# Autodesk Inventor assembly: electronic_board
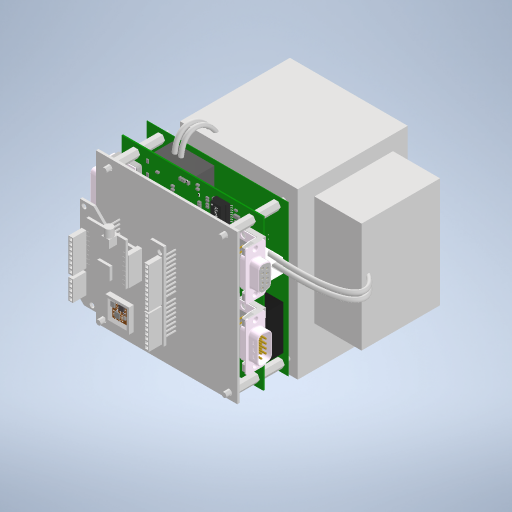
[picture p0: Inventor's stored thumbnail of the model, 512x512]
Saved by Autodesk Inventor 2023 (Build 270158000, 158)
## iProperties
Created: 2023-03-23
Part Number: electronic_board
Document SubType Name: Assembly
Designer: 310611102
Author: 310611102
## Documents named in this file (9)
- C:\Users\310611102\Documents\Inventor\SSR\avionics_2023ver\electronics\electronic_board.iam
- C:\Users\310611102\Documents\Inventor\SSR\avionics_2023ver\electronics\STM32 Communication Board ver1.0.ipt
- C:\Users\310611102\Documents\Inventor\SSR\avionics_2023ver\electronics\Power supply board.ipt
- C:\Users\310611102\Documents\Inventor\SSR\avionics_2023ver\electronics\copper_pillar_M3_L15.ipt
- C:\Users\310611102\Documents\Inventor\SSR\avionics_2023ver\electronics\battery_24V.ipt
- C:\Users\310611102\Documents\Inventor\SSR\avionics_2023ver\electronics\battery_5V.ipt
- C:\Users\310611102\Documents\Inventor\SSR\avionics_2023ver\electronics\MTI-7\MTi 1-series v3.iam
- C:\Users\310611102\Documents\Inventor\SSR\avionics_2023ver\electronics\LoRa_board.ipt
- C:\Users\310611102\Documents\Inventor\SSR\avionics_2023ver\electronics\empty_board.ipt
## Components (15 placed, 8 different names)
1. STM32 Communication Board ver1.0:1 — Insert:1, Insert:4, Insert:5
2. Power supply board:1 — Insert:2, Insert:3, Mate:1, Mate:2, Mate:3, Mate:4, Mate:5, Mate:6
3. battery_24V:1 — Mate:1, Flush:1, Mate:6
4. battery_5V:1 — Mate:2, Flush:1
5. MTi 1-series v3:1 [sub-assembly]
6. LoRa_board:1 — Mate:3, Mate:4, Mate:5
7. empty_board:1 — Insert:6, Insert:7
8. copper_pillar_M3_L15:1 — Insert:1, Insert:2
9. copper_pillar_M3_L15:2
10. copper_pillar_M3_L15:3 — Insert:3
11. copper_pillar_M3_L15:4
12. copper_pillar_M3_L15:5 — Insert:4, Insert:7
13. copper_pillar_M3_L15:6 — Insert:6
14. copper_pillar_M3_L15:7 — Insert:5
15. copper_pillar_M3_L15:8
## Component patterns: (2 elements, first: copper_pillar_M3_L15:1), (2 elements, first: copper_pillar_M3_L15:3), (2 elements, first: copper_pillar_M3_L15:5), (2 elements, first: copper_pillar_M3_L15:7)
## Relationships (14: Insert 7, Mate 6, Flush 1)
- Insert:1: STM32 Communication Board ver1.0:1 ↔ copper_pillar_M3_L15:1
- Insert:2: Power supply board:1 ↔ copper_pillar_M3_L15:1
- Insert:3: Power supply board:1 ↔ copper_pillar_M3_L15:3
- Mate:1 (10 mm): Power supply board:1 ↔ battery_24V:1
- Mate:2 (5 mm): Power supply board:1 ↔ battery_5V:1
- Flush:1: battery_24V:1 ↔ battery_5V:1
- Mate:3: Power supply board:1 ↔ LoRa_board:1
- Mate:4: Power supply board:1 ↔ LoRa_board:1
- Mate:5: Power supply board:1 ↔ LoRa_board:1
- Mate:6: Power supply board:1 ↔ battery_24V:1
- Insert:4: STM32 Communication Board ver1.0:1 ↔ copper_pillar_M3_L15:5
- Insert:5: STM32 Communication Board ver1.0:1 ↔ copper_pillar_M3_L15:7
- Insert:6: empty_board:1 ↔ copper_pillar_M3_L15:6
- Insert:7: empty_board:1 ↔ copper_pillar_M3_L15:5
